# Autodesk Inventor assembly: Mandy
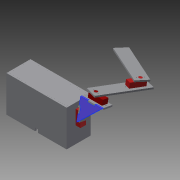
[picture p0: Inventor's stored thumbnail of the model, 180x180]
Saved by Autodesk Inventor 2013 (Build 170138000, 138)
## iProperties
Created: 2013-04-20
Part Number: Mandy
Document SubType Name: Assembly
Designer: fuji
Author: fuji
## Documents named in this file (10)
- C:\dev\p4\inventor\Mandy\Mandy.iam
- C:\dev\p4\inventor\Mandy\Top.ipt
- C:\dev\p4\inventor\Mandy\Front.ipt
- C:\dev\p4\inventor\Mandy\Side.ipt
- C:\dev\p4\inventor\Mandy\Servo.ipt
- C:\dev\p4\inventor\Mandy\AngleLower.ipt
- C:\dev\p4\inventor\Mandy\AngleTop.ipt
- C:\dev\p4\inventor\Mandy\UpperArm.ipt
- C:\dev\p4\inventor\Mandy\LowerArm.ipt
- C:\dev\p4\inventor\Mandy\AngleSide.ipt
## Components (13 placed, 9 different names)
1. Top:1 — Mate:1, Mate:2, Mate:3, Mate:4, Mate:5, Mate:6, Mate:7
2. Front:1 — Mate:1, Mate:2, Mate:5, Mate:8, Mate:10, Mate:11, Mate:12
3. Front:2 — Mate:3, Mate:4, Mate:6, Mate:9
4. Side:1 — Mate:7, Mate:8, Mate:9, Mate:13, Mate:14, Flush:1
5. Side:2 — Mate:10, Mate:11, Mate:12
6. Servo:1 — Mate:13, Mate:14, Flush:1, Insert:1
7. AngleLower:1 — Insert:1, Mate:15, Mate:16, Mate:17, Mate:24
8. AngleTop:1 — Mate:15, Mate:16, Mate:17, Mate:18, Mate:19, Flush:2, Mate:22, Mate:23
9. Servo:2 — Mate:18, Mate:19, Flush:2, Insert:2
10. UpperArm:1 — Insert:2, Mate:20, Mate:21, Flush:3
11. Servo:3 — Mate:20, Mate:21, Flush:3, Insert:3
12. LowerArm:1 — Insert:3
13. AngleSide:1 — Mate:22, Mate:23, Mate:24
## Relationships (30: Mate 24, Flush 3, Insert 3)
- Mate:1: Top:1 ↔ Front:1
- Mate:2: Top:1 ↔ Front:1
- Mate:3: Top:1 ↔ Front:2
- Mate:4: Top:1 ↔ Front:2
- Mate:5: Top:1 ↔ Front:1
- Mate:6: Top:1 ↔ Front:2
- Mate:7: Top:1 ↔ Side:1
- Mate:8: Front:1 ↔ Side:1
- Mate:9: Front:2 ↔ Side:1
- Mate:10: Front:1 ↔ Side:2
- Mate:11: Front:1 ↔ Side:2
- Mate:12: Front:1 ↔ Side:2
- Mate:13: Side:1 ↔ Servo:1
- Mate:14: Side:1 ↔ Servo:1
- Flush:1: Side:1 ↔ Servo:1
- Insert:1: Servo:1 ↔ AngleLower:1
- Mate:15: AngleLower:1 ↔ AngleTop:1
- Mate:16: AngleLower:1 ↔ AngleTop:1
- Mate:17: AngleLower:1 ↔ AngleTop:1
- Mate:18: AngleTop:1 ↔ Servo:2
- Mate:19: AngleTop:1 ↔ Servo:2
- Flush:2: AngleTop:1 ↔ Servo:2
- Insert:2: Servo:2 ↔ UpperArm:1
- Mate:20: UpperArm:1 ↔ Servo:3
- Mate:21: UpperArm:1 ↔ Servo:3
- Flush:3: UpperArm:1 ↔ Servo:3
- Insert:3: Servo:3 ↔ LowerArm:1
- Mate:22: AngleTop:1 ↔ AngleSide:1
- Mate:23: AngleTop:1 ↔ AngleSide:1
- Mate:24: AngleLower:1 ↔ AngleSide:1
